# Autodesk Inventor assembly: KabineKomplett
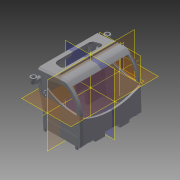
[picture p0: Inventor's stored thumbnail of the model, 180x180]
Saved by Autodesk Inventor 2015 (Build 190159000, 159)
## iProperties
Created: 2018-12-19
Part Number: KabineKomplett
Document SubType Name: Assembly
Designer: Boris
Author: Boris
## Documents named in this file (4)
- D:\Wisag Hiserv\HiSERV Smart Drive\WorkOrder\3D - Teile\KabineKomplett.iam
- D:\Wisag Hiserv\HiSERV Smart Drive\WorkOrder\3D - Teile\KabineTeil1.ipt
- D:\Wisag Hiserv\HiSERV Smart Drive\WorkOrder\3D - Teile\KabineTürLinksRechts.ipt
- D:\Wisag Hiserv\HiSERV Smart Drive\WorkOrder\3D - Teile\KabineTürLinksRechts_MIR.ipt
## Components (3 placed, 3 different names)
1. KabineTeil1:1 — Einfügen:1
2. KabineTürLinksRechts:1 — Einfügen:1
3. KabineTürLinksRechts_MIR:1
## Relationships (1: Insert 1)
- Einfügen:1 [Insert] (-3 mm): KabineTeil1:1 ↔ KabineTürLinksRechts:1
